# Autodesk Inventor assembly: LowerBackLink
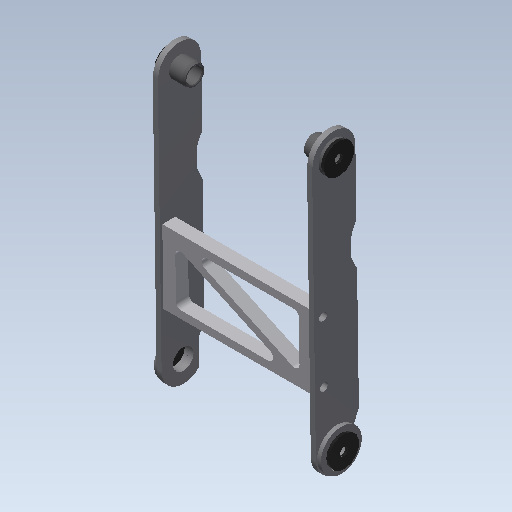
[picture p0: Inventor's stored thumbnail of the model, 512x512]
Saved by Autodesk Inventor 2020 (Build 240168000, 168)
## iProperties
Created: 2016-08-23
Part Number: LowerBackLink
Material: 一般
Document SubType Name: Assembly
Designer: hiro
Mass: 25.265 g
Surface Area: 146.992 cm^2
Volume: 11.3922 cm^3
Density: 2.21774 g/cm^3
Author: hiro
## Documents named in this file (6)
- C:\Users\Masato\Desktop\最新版\OpenPlatform_ver3_0\下半身\リンク\LowerBackLink.iam
- C:\Users\Masato\Desktop\最新版\OpenPlatform_ver3_0\下半身\リンク\リンク_メインフレーム_6_1.ipt
- C:\Users\Masato\Desktop\最新版\OpenPlatform_ver3_0\下半身\リンク\リンク_ふくらはぎ_サブフレーム_1_2.ipt
- C:\Users\Masato\Desktop\最新版\OpenPlatform_ver3_0\Ready_Made\80F-0608.ipt
- C:\Users\Masato\Desktop\最新版\OpenPlatform_ver3_0\Ready_Made\UUW-0312-10BH.ipt
- C:\Users\Masato\Desktop\最新版\OpenPlatform_ver3_0\Ready_Made\LFW-0815.ipt
## Components (11 placed, 5 different names)
1. リンク_ふくらはぎ_サブフレーム_1_2(予備案):1 — 挿入:2, 挿入:4, 挿入:11, 挿入:12
2. リンク_メインフレーム_6_1:1 — 挿入:2, 挿入:11, 挿入:14, 挿入:17
3. リンク_メインフレーム_6_1:2 — 挿入:4, 挿入:12, 挿入:13, 挿入:18
4. 80F-0608:1 — 挿入:13, 挿入:16
5. 80F-0608:2 — 挿入:14, 挿入:15
6. UUW-0312-10BH:1 — 挿入:15
7. UUW-0312-10BH:2 — 挿入:16
8. UUW-0312-10BH:3 — 挿入:20
9. UUW-0312-10BH:4 — 挿入:19
10. LFW-0815:1 — 挿入:18, 挿入:20
11. LFW-0815:2 — 挿入:17, 挿入:19
## Relationships (12: Insert 12)
- 挿入:2 [Insert]: リンク_ふくらはぎ_サブフレーム_1_2(予備案):1 ↔ リンク_メインフレーム_6_1:1
- 挿入:4 [Insert]: リンク_ふくらはぎ_サブフレーム_1_2(予備案):1 ↔ リンク_メインフレーム_6_1:2
- 挿入:11 [Insert]: リンク_ふくらはぎ_サブフレーム_1_2(予備案):1 ↔ リンク_メインフレーム_6_1:1
- 挿入:12 [Insert]: リンク_ふくらはぎ_サブフレーム_1_2(予備案):1 ↔ リンク_メインフレーム_6_1:2
- 挿入:13 [Insert]: リンク_メインフレーム_6_1:2 ↔ 80F-0608:1
- 挿入:14 [Insert]: リンク_メインフレーム_6_1:1 ↔ 80F-0608:2
- 挿入:15 [Insert]: 80F-0608:2 ↔ UUW-0312-10BH:1
- 挿入:16 [Insert]: 80F-0608:1 ↔ UUW-0312-10BH:2
- 挿入:17 [Insert]: リンク_メインフレーム_6_1:1 ↔ LFW-0815:2
- 挿入:18 [Insert]: リンク_メインフレーム_6_1:2 ↔ LFW-0815:1
- 挿入:19 [Insert]: UUW-0312-10BH:4 ↔ LFW-0815:2
- 挿入:20 [Insert]: UUW-0312-10BH:3 ↔ LFW-0815:1
